# Autodesk Inventor assembly: PrintedPully
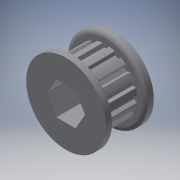
[picture p0: Inventor's stored thumbnail of the model, 180x180]
Saved by Autodesk Inventor 2019 (Build 230136000, 136)
## iProperties
Created: 2019-02-15
Part Number: PrintedPully
Document SubType Name: Assembly
Designer: james
Author: james
## Documents named in this file (3)
- F:\JimsDesign\2019CHS4089\PrintedPully.iam
- F:\JimsDesign\2019CHS4089\PullyShell1.ipt
- F:\JimsDesign\2019CHS4089\PullyHex.ipt
## Components (2 placed, 2 different names)
1. PullyShell1:1 — Mate:1, Flush:1
2. PullyHex:1 — Mate:1, Flush:1
## Relationships (2: Mate 1, Flush 1)
- Mate:1: PullyShell1:1 ↔ PullyHex:1
- Flush:1: PullyShell1:1 ↔ PullyHex:1
